# Autodesk Inventor assembly: BoltWasher4x8
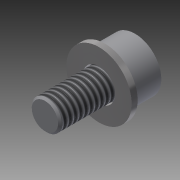
[picture p0: Inventor's stored thumbnail of the model, 180x180]
Saved by Autodesk Inventor 2015 SP1 (Build 190203100, 203)
## iProperties
Category: Hardware
Created: 2015-02-01
Part Number: BoltWasher4x8
Document SubType Name: Assembly
Designer: Jack
Vendor: Misumi
Author: Jack
Title: Bolt + Washer SHCS4x8
## Documents named in this file (3)
- C:\Users\Jack\ownCloud\Projects\CoreXY\InventorModel\Hardware\BoltWashers\BoltWasher4\BoltWasher4x8.iam
- C:\Users\Jack\ownCloud\Projects\CoreXY\InventorModel\Hardware\Bolts\SHCS\SHCS4\SHCS4x8.ipt
- C:\Users\Jack\ownCloud\Projects\CoreXY\InventorModel\Hardware\Wahsers\M4Washer.ipt
## Components (2 placed, 2 different names)
1. SHCS4x8:1 — Mate:1, Mate:2
2. M4Washer:1 — Mate:1, Mate:2
## Relationships (2: Mate 2)
- Mate:1: SHCS4x8:1 ↔ M4Washer:1
- Mate:2: SHCS4x8:1 ↔ M4Washer:1
